# Autodesk Inventor assembly: ensamblaje gramera
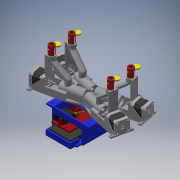
[picture p0: Inventor's stored thumbnail of the model, 180x180]
Saved by Autodesk Inventor 2019 (Build 230136000, 136)
## iProperties
Created: 2019-10-01
Part Number: ensamblaje gramera
Document SubType Name: Assembly
Designer: dbrau
Author: dbrau
## Documents named in this file (12)
- D:\U\Semestre III mecánica\seminario\ensamblaje gramera.iam
- D:\U\Semestre III mecánica\seminario\hs-311_asm.ipt
- D:\U\Semestre III mecánica\seminario\gramera.ipt
- D:\U\Semestre III mecánica\seminario\soporte_carga.ipt
- D:\U\Semestre III mecánica\seminario\soporte_gramera2.ipt
- D:\U\Semestre III mecánica\seminario\conten_elem_solidos.ipt
- D:\U\Semestre III mecánica\seminario\viela_gramera.ipt
- D:\U\Semestre III mecánica\seminario\SoporteDispensadorParticulas v7.ipt
- D:\U\Semestre III mecánica\seminario\NEMA 17 with T5 Pulley.iam
- D:\U\Semestre III mecánica\seminario\union_botella.ipt
- D:\U\Semestre III mecánica\seminario\perilla.ipt
- D:\U\Semestre III mecánica\seminario\valvula.ipt
## Components (24 placed, 11 different names)
1. hs-311_asm:1 — Insert:3
2. gramera:1 — Mate:1, Mate:2, Mate:3, Mate:5
3. soporte_carga:1 — Mate:1, Mate:2, Mate:3, Mate:4, Flush:1, Flush:2, Mate:8, Mate:9, Mate:11
4. soporte_gramera2:1 — Mate:4, Mate:5, Mate:6, Mate:7, Flush:1
5. conten_elem_solidos:1 — Mate:6, Mate:7
6. viela_gramera:1 — Insert:3
7. SoporteDispensadorParticulas v7:1 — Mate:10, Flush:3, Mate:11, Insert:4, Insert:5, Insert:6, Insert:7, Insert:12, Insert:13
8. SoporteDispensadorParticulas v7:2 — Flush:2, Mate:8, Mate:9, Mate:10, Flush:3, Insert:8, Insert:9, Insert:10, Insert:11, Insert:14, Insert:15
9. NEMA 17 with T5 Pulley:1 [sub-assembly] — Insert:4, Insert:5
10. NEMA 17 with T5 Pulley:2 [sub-assembly] — Insert:8, Insert:9
11. NEMA 17 with T5 Pulley:3 [sub-assembly] — Insert:10, Insert:11
12. NEMA 17 with T5 Pulley:4 [sub-assembly] — Insert:6, Insert:7
13. union_botella:1 — Insert:12, Cylindrical:1, Cylindrical:7
14. union_botella:2 — Insert:13, Cylindrical:2, Cylindrical:6
15. union_botella:3 — Insert:14, Cylindrical:3, Cylindrical:5
16. union_botella:4 — Insert:15, Cylindrical:4, Cylindrical:8
17. perilla:1 — Cylindrical:1
18. perilla:2 — Cylindrical:2
19. perilla:3 — Cylindrical:3
20. perilla:4 — Cylindrical:4
21. valvula:1 — Cylindrical:7
22. valvula:2 — Cylindrical:5
23. valvula:3 — Cylindrical:8
24. valvula:4 — Cylindrical:6
## Relationships (35: Insert 13, Mate 11, CylindricalJoint 8, Flush 3)
- Mate:1 (11.3 mm): gramera:1 ↔ soporte_carga:1
- Mate:2: gramera:1 ↔ soporte_carga:1
- Mate:3 (0.2 mm): gramera:1 ↔ soporte_carga:1
- Mate:4 (0.1 mm): soporte_carga:1 ↔ soporte_gramera2:1
- Mate:5 (0.1 mm): gramera:1 ↔ soporte_gramera2:1
- Mate:6 (0.1 mm): soporte_gramera2:1 ↔ conten_elem_solidos:1
- Mate:7 (0.1 mm): soporte_gramera2:1 ↔ conten_elem_solidos:1
- Insert:3: hs-311_asm:1 ↔ viela_gramera:1
- Flush:1 (-34.5 mm): soporte_carga:1 ↔ soporte_gramera2:1
- Flush:2 (5.52 mm): soporte_carga:1 ↔ SoporteDispensadorParticulas v7:2
- Mate:8: soporte_carga:1 ↔ SoporteDispensadorParticulas v7:2
- Mate:9 (-73.95 mm): soporte_carga:1 ↔ SoporteDispensadorParticulas v7:2
- Mate:10: SoporteDispensadorParticulas v7:1 ↔ SoporteDispensadorParticulas v7:2
- Flush:3: SoporteDispensadorParticulas v7:1 ↔ SoporteDispensadorParticulas v7:2
- Mate:11: soporte_carga:1 ↔ SoporteDispensadorParticulas v7:1
- Insert:4: SoporteDispensadorParticulas v7:1 ↔ NEMA 17 with T5 Pulley:1
- Insert:5: SoporteDispensadorParticulas v7:1 ↔ NEMA 17 with T5 Pulley:1
- Insert:6: SoporteDispensadorParticulas v7:1 ↔ NEMA 17 with T5 Pulley:4
- Insert:7: SoporteDispensadorParticulas v7:1 ↔ NEMA 17 with T5 Pulley:4
- Insert:8: SoporteDispensadorParticulas v7:2 ↔ NEMA 17 with T5 Pulley:2
- Insert:9: SoporteDispensadorParticulas v7:2 ↔ NEMA 17 with T5 Pulley:2
- Insert:10: SoporteDispensadorParticulas v7:2 ↔ NEMA 17 with T5 Pulley:3
- Insert:11: SoporteDispensadorParticulas v7:2 ↔ NEMA 17 with T5 Pulley:3
- Insert:12: SoporteDispensadorParticulas v7:1 ↔ union_botella:1
- Insert:13: SoporteDispensadorParticulas v7:1 ↔ union_botella:2
- Insert:14: SoporteDispensadorParticulas v7:2 ↔ union_botella:3
- Insert:15: SoporteDispensadorParticulas v7:2 ↔ union_botella:4
- Cylindrical:1: union_botella:1 ↔ perilla:1
- Cylindrical:2: union_botella:2 ↔ perilla:2
- Cylindrical:3: union_botella:3 ↔ perilla:3
- Cylindrical:4: union_botella:4 ↔ perilla:4
- Cylindrical:5: union_botella:3 ↔ valvula:2
- Cylindrical:6: union_botella:2 ↔ valvula:4
- Cylindrical:7: union_botella:1 ↔ valvula:1
- Cylindrical:8: union_botella:4 ↔ valvula:3
